# Autodesk Inventor assembly: nhk36
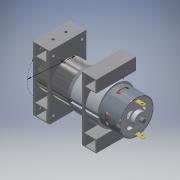
[picture p0: Inventor's stored thumbnail of the model, 180x180]
Saved by Autodesk Inventor 2019 (Build 230136000, 136)
## iProperties
Created: 2022-02-27
Part Number: nhk36
Material: 一般
Document SubType Name: Assembly
Designer: yuta
Author: yuta
## Documents named in this file (7)
- C:\Users\yuta\Documents\NHK\nhk36.iam
- C:\Users\yuta\Documents\NHK\nhk28.ipt
- C:\Users\yuta\Documents\NHK\nhk29.ipt
- C:\Users\yuta\Documents\NHK\RS775+gennsoku.iam
- C:\Users\yuta\Documents\NHK\nhk30.ipt
- C:\Users\yuta\Documents\NHK\nhk31.ipt
- C:\Users\yuta\Documents\NHK\nhk32.ipt
## Components (8 placed, 6 different names)
1. nhk28:1 — メイト:1, フラッシュ:1, フラッシュ:2, メイト:2, フラッシュ:3, フラッシュ:4, メイト:3, フラッシュ:5
2. nhk29:1 — メイト:2, フラッシュ:3, フラッシュ:4
3. nhk29:2 — メイト:1, フラッシュ:1, フラッシュ:2, メイト:4, メイト:6
4. RS775+gennsoku:1 [sub-assembly] — メイト:3, フラッシュ:5, メイト:5, フラッシュ:6
5. nhk30:1 — メイト:4, メイト:6
6. nhk31:1 — メイト:5, フラッシュ:6, フラッシュ:7, メイト:7, フラッシュ:8, フラッシュ:9, メイト:8, フラッシュ:10
7. nhk32:2 — フラッシュ:7, メイト:7, フラッシュ:8
8. nhk32:3 — フラッシュ:9, メイト:8, フラッシュ:10
## Relationships (18: Flush 10, Mate 8)
- メイト:1 [Mate]: nhk28:1 ↔ nhk29:2
- フラッシュ:1 [Flush]: nhk28:1 ↔ nhk29:2
- フラッシュ:2 [Flush]: nhk28:1 ↔ nhk29:2
- メイト:2 [Mate]: nhk28:1 ↔ nhk29:1
- フラッシュ:3 [Flush]: nhk28:1 ↔ nhk29:1
- フラッシュ:4 [Flush]: nhk28:1 ↔ nhk29:1
- メイト:3 [Mate]: nhk28:1 ↔ RS775+gennsoku:1
- フラッシュ:5 [Flush]: nhk28:1 ↔ RS775+gennsoku:1
- メイト:4 [Mate]: nhk29:2 ↔ nhk30:1
- メイト:5 [Mate]: RS775+gennsoku:1 ↔ nhk31:1
- フラッシュ:6 [Flush] (15 mm): RS775+gennsoku:1 ↔ nhk31:1
- メイト:6 [Mate]: nhk29:2 ↔ nhk30:1
- フラッシュ:7 [Flush]: nhk31:1 ↔ nhk32:2
- メイト:7 [Mate]: nhk31:1 ↔ nhk32:2
- フラッシュ:8 [Flush]: nhk31:1 ↔ nhk32:2
- フラッシュ:9 [Flush]: nhk31:1 ↔ nhk32:3
- メイト:8 [Mate]: nhk31:1 ↔ nhk32:3
- フラッシュ:10 [Flush]: nhk31:1 ↔ nhk32:3
